# Autodesk Inventor assembly: s-assy-HBLFSN5h5
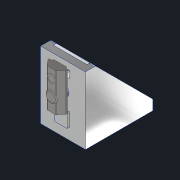
[picture p0: Inventor's stored thumbnail of the model, 180x180]
Saved by Autodesk Inventor 2022 (Build 260153000, 153)
## iProperties
Created: 2021-10-04
Part Number: s-assy-HBLFSN5h5
Document SubType Name: Assembly
Designer: Yuta Kage
Mass: 29.4309 g
Surface Area: 60.6911 cm^2
Volume: 7.81384 cm^3
Density: 3.76652 g/cm^3
Author: Yuta Kage
## Documents named in this file (4)
- G:\その他のパソコン\ZephyrusG14\Desktop\proj-catchrobo2022\assy-catchrobo2022\s-assy-HBLFSN5h5.iam
- G:\その他のパソコン\ZephyrusG14\Desktop\proj-catchrobo2022\assy-catchrobo2022\HBLFSN5h5.ipt
- G:\その他のパソコン\ZephyrusG14\Desktop\proj-catchrobo2022\assy-catchrobo2022\CB5_10.ipt
- G:\その他のパソコン\ZephyrusG14\Desktop\proj-catchrobo2022\assy-catchrobo2022\HNTP5-5.ipt
## Components (5 placed, 3 different names)
1. HBLFSN5h5:1 — メイト:5, メイト:6, メイト:7, メイト:8, メイト:11, メイト:12
2. CB5_10:1 — メイト:5, メイト:6, メイト:9
3. CB5_10:2 — メイト:7, メイト:8, メイト:10
4. HNTP5-5:1 — メイト:9, メイト:12, メイト:13
5. HNTP5-5:2 — メイト:10, メイト:11, フラッシュ:1
## Relationships (10: Mate 9, Flush 1)
- メイト:5 [Mate]: HBLFSN5h5:1 ↔ CB5_10:1
- メイト:6 [Mate]: HBLFSN5h5:1 ↔ CB5_10:1
- メイト:7 [Mate]: HBLFSN5h5:1 ↔ CB5_10:2
- メイト:8 [Mate]: HBLFSN5h5:1 ↔ CB5_10:2
- メイト:9 [Mate]: CB5_10:1 ↔ HNTP5-5:1
- メイト:10 [Mate]: CB5_10:2 ↔ HNTP5-5:2
- メイト:11 [Mate] (2 mm): HBLFSN5h5:1 ↔ HNTP5-5:2
- メイト:12 [Mate] (2 mm): HBLFSN5h5:1 ↔ HNTP5-5:1
- メイト:13 [Mate]: HNTP5-5:1
- フラッシュ:1 [Flush]: HNTP5-5:2
